# Autodesk Inventor assembly: two_wheels
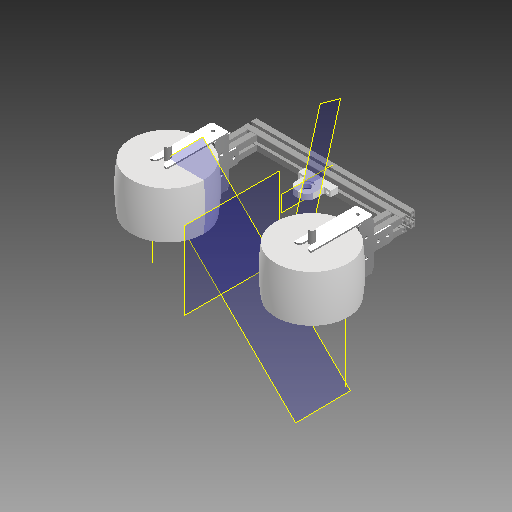
[picture p0: Inventor's stored thumbnail of the model, 512x512]
Saved by Autodesk Inventor 2021.3 (Build 253353000, 353)
## iProperties
Created: 2021-05-27
Part Number: two_wheels
Document SubType Name: Assembly
Designer: gisen
Author: gisen
## Documents named in this file (6)
- C:\Users\gisen\workspace\beetle_inventor_model\suspension\bogie.iam
- C:\Users\gisen\workspace\beetle_inventor_model\suspension\wheel_with_mounts.iam
- C:\Users\gisen\workspace\beetle_inventor_model\suspension\C-BGHKA6902ZZ-30\C-BGHKA6902ZZ-30.iam
- C:\Users\gisen\workspace\beetle_inventor_model\suspension\frame\AFS-3030-60.ipt
- C:\Users\gisen\workspace\beetle_inventor_model\suspension\frame\AFS-3030-330.ipt
- C:\Users\gisen\workspace\beetle_inventor_model\suspension\CAM\wheel_frame_mount_short.ipt
## Components (8 placed, 5 different names)
1. wheel_with_mounts:1 [sub-assembly] — メイト:18, フラッシュ:19, フラッシュ:28, メイト:29, メイト:30, メイト:33
2. C-BGHKA6902ZZ-30:1 [sub-assembly] — メイト:38, メイト:39, メイト:40, メイト:41
3. AFS-3030-60:1 — フラッシュ:24, メイト:27, フラッシュ:25, フラッシュ:26, フラッシュ:27, メイト:36, メイト:37, フラッシュ:30, 対称度:1
4. AFS-3030-60:2 — フラッシュ:24, メイト:28, フラッシュ:25, メイト:31, メイト:32, メイト:33, 対称度:1
5. AFS-3030-330:1 — メイト:27, メイト:28, フラッシュ:26, フラッシュ:27, メイト:38, メイト:39, メイト:40
6. wheel_frame_mount:1 — フラッシュ:28, メイト:29, メイト:30, メイト:31, メイト:32
7. wheel_with_mounts:2 [sub-assembly] — メイト:36, メイト:37, フラッシュ:30, フラッシュ:31
8. wheel_frame_mount:2
## Relationships (32: Mate 22, Flush 9, Symmetry 1)
- メイト:10 [Mate]
- メイト:11 [Mate]
- メイト:12 [Mate]
- メイト:13 [Mate]
- メイト:14 [Mate] (200 mm)
- メイト:16 [Mate]
- メイト:18 [Mate]: wheel_with_mounts:1
- フラッシュ:19 [Flush]: wheel_with_mounts:1
- フラッシュ:24 [Flush]: AFS-3030-60:1 ↔ AFS-3030-60:2
- メイト:27 [Mate]: AFS-3030-60:1 ↔ AFS-3030-330:1
- メイト:28 [Mate]: AFS-3030-60:2 ↔ AFS-3030-330:1
- フラッシュ:25 [Flush]: AFS-3030-60:1 ↔ AFS-3030-60:2
- フラッシュ:26 [Flush]: AFS-3030-60:1 ↔ AFS-3030-330:1
- フラッシュ:27 [Flush]: AFS-3030-60:1 ↔ AFS-3030-330:1
- フラッシュ:28 [Flush]: wheel_with_mounts:1 ↔ wheel_frame_mount:1
- メイト:29 [Mate]: wheel_with_mounts:1 ↔ wheel_frame_mount:1
- メイト:30 [Mate]: wheel_with_mounts:1 ↔ wheel_frame_mount:1
- メイト:31 [Mate]: AFS-3030-60:2 ↔ wheel_frame_mount:1
- メイト:32 [Mate] (-15 mm): AFS-3030-60:2 ↔ wheel_frame_mount:1
- メイト:33 [Mate]: wheel_with_mounts:1 ↔ AFS-3030-60:2
- [Flush]: wheel_with_mounts:2 ↔ wheel_frame_mount:2
- [Mate]: wheel_with_mounts:2 ↔ wheel_frame_mount:2
- [Mate]: wheel_with_mounts:2 ↔ wheel_frame_mount:2
- メイト:36 [Mate]: AFS-3030-60:1 ↔ wheel_with_mounts:2
- メイト:37 [Mate]: AFS-3030-60:1 ↔ wheel_with_mounts:2
- フラッシュ:30 [Flush]: AFS-3030-60:1 ↔ wheel_with_mounts:2
- 対称度:1 [Symmetry]: AFS-3030-60:1 ↔ AFS-3030-60:2
- メイト:38 [Mate]: C-BGHKA6902ZZ-30:1 ↔ AFS-3030-330:1
- メイト:39 [Mate] (-15 mm): C-BGHKA6902ZZ-30:1 ↔ AFS-3030-330:1
- メイト:40 [Mate] (-15 mm): C-BGHKA6902ZZ-30:1 ↔ AFS-3030-330:1
- メイト:41 [Mate]: C-BGHKA6902ZZ-30:1
- フラッシュ:31 [Flush]: wheel_with_mounts:2
## Named parameters: wheel_base = 400 mm, d73_d67 = 0 mm, d74_d68 = 0 mm, d75_d69 = 0 mm
